# Autodesk Inventor assembly: UR5 with not hand
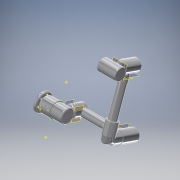
[picture p0: Inventor's stored thumbnail of the model, 180x180]
Saved by Autodesk Inventor 2016 (Build 200138000, 138)
## iProperties
Created: 2017-12-24
Part Number: UR5 with not hand
Document SubType Name: Assembly
Designer: kornbot
Author: kornbot
## Documents named in this file (10)
- C:\Users\kornbot\Documents\UR5 with not hand.iam
- C:\Users\kornbot\Documents\UR5 Joint base connection.ipt
- C:\Users\kornbot\Documents\UR5 base2.ipt
- C:\Users\kornbot\Documents\UR5 upper joint shoulder.ipt
- C:\Users\kornbot\Documents\UR5 joint shoulder 2.ipt
- C:\Users\kornbot\Documents\UR5 extended arm.ipt
- C:\Users\kornbot\Documents\UR5 joint elbow2.ipt
- C:\Users\kornbot\Documents\UR5 joint elbow3.ipt
- C:\Users\kornbot\Documents\UR5 Joint to wrist.ipt
- C:\Users\kornbot\Documents\UR5 End to wrist.ipt
## Components (12 placed, 9 different names)
1. UR5 base2:1 — Rotational:1
2. UR5 Joint base connection:1 — Rotational:1, Rigid:1, Rigid:2
3. UR5 Joint base connection:2 — Rigid:1
4. UR5 upper joint shoulder:1 — Rigid:2, Rotational:2
5. UR5 joint shoulder 2:1 — Rotational:2, Rigid:3
6. UR5 joint shoulder 2:2 — Rigid:3, Rotational:3
7. UR5 extended arm:1 — Rotational:3, Rigid:4
8. UR5 joint elbow3:1 — Rigid:4, Rotational:4
9. UR5 Joint to wrist:1 — Rotational:4, Rigid:5
10. UR5 End to wrist:1 — Rigid:5, Rigid:6
11. UR5 joint elbow2:1 — Rigid:6, Rotational:5
12. UR5 joint elbow2:2 — Rotational:5
## Relationships (11: WeldJoint 6, RevoluteJoint 5)
- Rotational:1 [RevoluteJoint]: UR5 base2:1 ↔ UR5 Joint base connection:1
- Rigid:1 [WeldJoint]: UR5 Joint base connection:1 ↔ UR5 Joint base connection:2
- Rigid:2 [WeldJoint]: UR5 Joint base connection:1 ↔ UR5 upper joint shoulder:1
- Rotational:2 [RevoluteJoint]: UR5 upper joint shoulder:1 ↔ UR5 joint shoulder 2:1
- Rigid:3 [WeldJoint]: UR5 joint shoulder 2:1 ↔ UR5 joint shoulder 2:2
- Rotational:3 [RevoluteJoint] (-9.25 mm): UR5 joint shoulder 2:2 ↔ UR5 extended arm:1
- Rigid:4 [WeldJoint] (21.75 mm): UR5 extended arm:1 ↔ UR5 joint elbow3:1
- Rotational:4 [RevoluteJoint]: UR5 joint elbow3:1 ↔ UR5 Joint to wrist:1
- Rigid:5 [WeldJoint]: UR5 Joint to wrist:1 ↔ UR5 End to wrist:1
- Rigid:6 [WeldJoint]: UR5 End to wrist:1 ↔ UR5 joint elbow2:1
- Rotational:5 [RevoluteJoint]: UR5 joint elbow2:1 ↔ UR5 joint elbow2:2
